# Autodesk Inventor assembly: Dough arm assembly
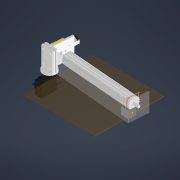
[picture p0: Inventor's stored thumbnail of the model, 180x180]
Saved by Autodesk Inventor 2021 (Build 250183000, 183)
## iProperties
Created: 2022-05-21
Part Number: Dough arm assembly
Document SubType Name: Assembly
Designer: techv
Author: techv
## Documents named in this file (9)
- D:\Projects\P_Baker Bot\Design\dough arm assembly\Dough arm assembly.iam
- D:\Projects\A_Electronics CAD model\TOWER PRO MG-995, ANALOG SERVO.ipt
- D:\Projects\P_Baker Bot\Design\dough arm assembly\poly carbonate plate.ipt
- D:\Projects\A_Electronics CAD model\BO DC Motor.ipt
- D:\Projects\P_Baker Bot\Design\dough arm assembly\arm - servo mount.ipt
- D:\Projects\P_Baker Bot\Design\dough arm assembly\arm1.ipt
- D:\Projects\P_Baker Bot\Design\dough arm assembly\arm2.ipt
- D:\Projects\P_Baker Bot\Design\dough arm assembly\l bracket.ipt
- D:\Projects\P_Baker Bot\Design\dough arm assembly\Roller.ipt
## Components (8 placed, 8 different names)
1. TOWER PRO MG-995, ANALOG SERVO:1 — Mate:1, Mate:2, Mate:5, Mate:6, Mate:7
2. poly carbonate plate:1 — Mate:2, Mate:5
3. BO DC Motor:1 — Mate:13, Mate:14, Mate:15, Flush:3
4. arm - servo mount:1 — Mate:6, Mate:7, Mate:8, Mate:13, Mate:14, Mate:15, Mate:16
5. arm1:1 — Flush:1, Mate:8, Mate:11, Mate:16
6. arm2:1 — Flush:1, Mate:12, Flush:2
7. l bracket:1 — Mate:11, Mate:12, Flush:2
8. Roller:1 — Flush:3
## Relationships (15: Mate 12, Flush 3)
- Mate:1: TOWER PRO MG-995, ANALOG SERVO:1
- Mate:2 (-5 mm): TOWER PRO MG-995, ANALOG SERVO:1 ↔ poly carbonate plate:1
- Mate:5 (10 mm): TOWER PRO MG-995, ANALOG SERVO:1 ↔ poly carbonate plate:1
- Flush:1: arm1:1 ↔ arm2:1
- Mate:6: TOWER PRO MG-995, ANALOG SERVO:1 ↔ arm - servo mount:1
- Mate:7: TOWER PRO MG-995, ANALOG SERVO:1 ↔ arm - servo mount:1
- Mate:8: arm - servo mount:1 ↔ arm1:1
- Mate:11: arm1:1 ↔ l bracket:1
- Mate:12: arm2:1 ↔ l bracket:1
- Mate:13: BO DC Motor:1 ↔ arm - servo mount:1
- Mate:14: BO DC Motor:1 ↔ arm - servo mount:1
- Flush:2 (-20 mm): arm2:1 ↔ l bracket:1
- Mate:15: BO DC Motor:1 ↔ arm - servo mount:1
- Flush:3: BO DC Motor:1 ↔ Roller:1
- Mate:16: arm - servo mount:1 ↔ arm1:1
